# Autodesk Inventor assembly: move_straight
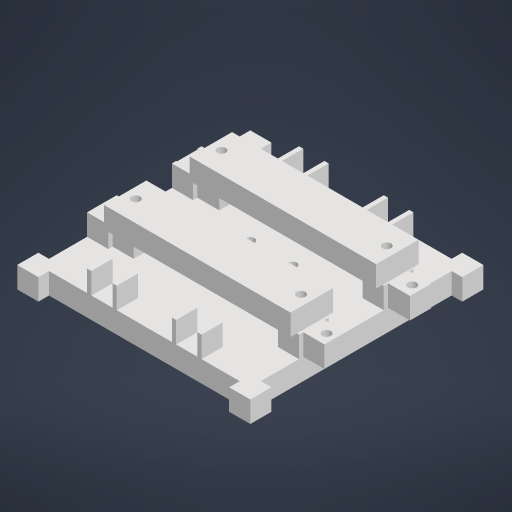
[picture p0: Inventor's stored thumbnail of the model, 512x512]
Saved by Autodesk Inventor 2024.3 (Build 283343000, 343)
## iProperties
Created: 2024-09-29
Part Number: move_straight
Document SubType Name: Assembly
Designer: sam
Author: sam
## Documents named in this file (4)
- N:\Cad\computer\gates\move_straight.iam
- N:\Cad\computer\gates\base.ipt
- N:\Cad\computer\gates\block.ipt
- N:\Cad\computer\gates\extender _med.ipt
## Components (7 placed, 3 different names)
1. base:1 — Mate:1, Mate:2, Mate:3, Mate:4, Mate:5, Mate:6, Mate:7, Mate:8
2. block:1 — Mate:2, Mate:6, Mate:13, Mate:16
3. block:2 — Mate:1, Mate:7, Mate:14, Mate:15
4. block:3 — Mate:3, Mate:8, Mate:10, Mate:11
5. block:4 — Mate:4, Mate:5, Mate:9, Mate:12
6. extender _med:1 — Mate:9, Mate:10, Mate:11, Mate:12
7. extender _med:2 — Mate:13, Mate:14, Mate:15, Mate:16
## Relationships (16: Mate 16)
- Mate:1: base:1 ↔ block:2
- Mate:2: base:1 ↔ block:1
- Mate:3: base:1 ↔ block:3
- Mate:4: base:1 ↔ block:4
- Mate:5: base:1 ↔ block:4
- Mate:6: base:1 ↔ block:1
- Mate:7: base:1 ↔ block:2
- Mate:8: base:1 ↔ block:3
- Mate:9: block:4 ↔ extender _med:1
- Mate:10: block:3 ↔ extender _med:1
- Mate:11: block:3 ↔ extender _med:1
- Mate:12: block:4 ↔ extender _med:1
- Mate:13: block:1 ↔ extender _med:2
- Mate:14: block:2 ↔ extender _med:2
- Mate:15: block:2 ↔ extender _med:2
- Mate:16: block:1 ↔ extender _med:2
